# Autodesk Inventor assembly: gear20
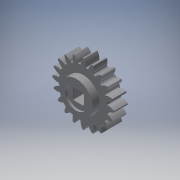
[picture p0: Inventor's stored thumbnail of the model, 180x180]
Saved by Autodesk Inventor 2019 (Build 230136000, 136)
## iProperties
Created: 2019-01-25
Part Number: gear20
Document SubType Name: Assembly
Designer: Varga Daniel
Author: Varga Daniel
## Documents named in this file (3)
- C:\!_Dani\!_cloud\OneDrive\!_munka\Revolution\RevvyDemoKit\Structural parts\Demo parts\Gears\gear20.iam
- C:\!_Dani\!_cloud\OneDrive\!_munka\Revolution\RevvyDemoKit\Structural parts\Demo parts\Gears\gear20.ipt
- C:\!_Dani\!_cloud\OneDrive\!_munka\Revolution\RevvyDemoKit\Structural parts\Demo parts\Gears\gear_collar_small.ipt
## Components (3 placed, 2 different names)
1. gear_collar_small:1 — Mate:1, Flush:1, Flush:2, Angle:1
2. gear20:1 — Mate:1, Mate:3, Angle:1
3. gear_collar_small:2 — Mate:3, Flush:1, Flush:2
## Relationships (5: Mate 2, Flush 2, Angle 1)
- Mate:1: gear_collar_small:1 ↔ gear20:1
- Mate:3: gear20:1 ↔ gear_collar_small:2
- Flush:1: gear_collar_small:1 ↔ gear_collar_small:2
- Flush:2: gear_collar_small:1 ↔ gear_collar_small:2
- Angle:1 (0 deg): gear_collar_small:1 ↔ gear20:1
